# Autodesk Inventor assembly: 09
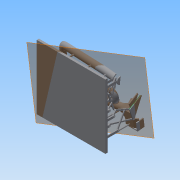
[picture p0: Inventor's stored thumbnail of the model, 180x180]
Saved by Autodesk Inventor 2015 (Build 190159000, 159)
## iProperties
Created: 2018-05-07
Part Number: 09
Document SubType Name: Assembly
Designer: 王博聖
Author: 王博聖
## Documents named in this file (14)
- C:\Users\王博聖\Desktop\0507\09.iam
- C:\Users\王博聖\Desktop\0507\0.ipt
- C:\Users\王博聖\Desktop\0507\1.ipt
- C:\Users\王博聖\Desktop\0507\1-1.ipt
- C:\Users\王博聖\Desktop\0507\1-2.ipt
- C:\Users\王博聖\Desktop\0507\1-3.ipt
- C:\Users\王博聖\Desktop\0507\1-4.ipt
- C:\Users\王博聖\Desktop\0507\2.ipt
- C:\Users\王博聖\Desktop\0507\3.ipt
- C:\Users\王博聖\Desktop\0507\4.ipt
- C:\Users\王博聖\Desktop\0507\5.ipt
- C:\Users\王博聖\Desktop\0507\4456.ipt
- C:\Users\王博聖\Desktop\0507\4444.ipt
- C:\Users\王博聖\Desktop\0507\66666.ipt
## Components (23 placed, 13 different names)
1. 0:1 — 貼合:1, 貼合:2, 貼合:3, 貼合:4, 貼合:5, 貼合:14, 旋轉:1, 齊平:2, 齊平:3, 齊平:5, 齊平:6, 齊平:7, 貼合:29, 齊平:9, 貼合:37, 貼合:38, 貼合:39
2. 1:1 — 貼合:1, 貼合:13, 貼合:25, 貼合:31, 齊平:11
3. 1-1:1 — 貼合:13, 貼合:15, 貼合:24, 貼合:25, 齊平:4, 貼合:33
4. 1-4:1 — 貼合:9, 貼合:20, 貼合:26, 貼合:27, 貼合:35, 貼合:36
5. 2:1 — 貼合:2, 貼合:16, 貼合:23, 貼合:30, 齊平:10
6. 3:1 — 貼合:3, 貼合:14, 貼合:18, 貼合:21, 旋轉:1, 貼合:28, 齊平:8
7. 4:1 — 貼合:4, 貼合:9, 貼合:26
8. 5:1 — 貼合:5, 貼合:19, 貼合:34
9. 1-2:1 — 貼合:15, 貼合:16, 貼合:17, 貼合:22, 貼合:23, 貼合:24, 貼合:32
10. 1-3:1 — 貼合:17, 貼合:18, 貼合:19, 貼合:20, 貼合:21, 貼合:22, 貼合:27
11. 4456:1 — 齊平:2, 齊平:3, 齊平:4, 齊平:5, 齊平:6, 齊平:7
12. 4444:1 — 貼合:32
13. 4444:2 — 貼合:33
14. 4444:3 — 貼合:30, 齊平:10
15. 4444:4 — 貼合:31, 齊平:11
16. 4444:5 — 貼合:29, 齊平:9
17. 4444:6 — 貼合:39
18. 4444:7 — 貼合:34
19. 4444:8 — 貼合:35
20. 4444:9 — 貼合:37
21. 4444:10 — 貼合:38
22. 4444:11 — 貼合:36
23. 66666:1 — 貼合:28, 齊平:8
## Relationships (44: Mate 33, Flush 10, RevoluteJoint 1)
- 貼合:1 [Mate]: 0:1 ↔ 1:1
- 貼合:2 [Mate]: 0:1 ↔ 2:1
- 貼合:3 [Mate]: 0:1 ↔ 3:1
- 貼合:4 [Mate]: 0:1 ↔ 4:1
- 貼合:5 [Mate]: 0:1 ↔ 5:1
- 貼合:9 [Mate]: 1-4:1 ↔ 4:1
- 貼合:13 [Mate]: 1:1 ↔ 1-1:1
- 貼合:14 [Mate]: 0:1 ↔ 3:1
- 貼合:15 [Mate]: 1-1:1 ↔ 1-2:1
- 貼合:16 [Mate]: 2:1 ↔ 1-2:1
- 貼合:17 [Mate]: 1-2:1 ↔ 1-3:1
- 貼合:18 [Mate]: 3:1 ↔ 1-3:1
- 貼合:19 [Mate]: 5:1 ↔ 1-3:1
- 貼合:20 [Mate]: 1-4:1 ↔ 1-3:1
- 貼合:21 [Mate]: 3:1 ↔ 1-3:1
- 貼合:22 [Mate]: 1-2:1 ↔ 1-3:1
- 貼合:23 [Mate]: 2:1 ↔ 1-2:1
- 貼合:24 [Mate]: 1-1:1 ↔ 1-2:1
- 貼合:25 [Mate]: 1:1 ↔ 1-1:1
- 貼合:26 [Mate]: 1-4:1 ↔ 4:1
- 貼合:27 [Mate]: 1-4:1 ↔ 1-3:1
- 旋轉:1 [RevoluteJoint]: 0:1 ↔ 3:1
- 齊平:2 [Flush]: 0:1 ↔ 4456:1
- 齊平:3 [Flush]: 0:1 ↔ 4456:1
- 齊平:4 [Flush]: 1-1:1 ↔ 4456:1
- 齊平:5 [Flush]: 0:1 ↔ 4456:1
- 齊平:6 [Flush] (-23 mm): 0:1 ↔ 4456:1
- 齊平:7 [Flush]: 0:1 ↔ 4456:1
- 貼合:28 [Mate]: 3:1 ↔ 66666:1
- 齊平:8 [Flush]: 3:1 ↔ 66666:1
- 貼合:29 [Mate]: 0:1 ↔ 4444:5
- 齊平:9 [Flush]: 0:1 ↔ 4444:5
- 貼合:30 [Mate]: 2:1 ↔ 4444:3
- 齊平:10 [Flush]: 2:1 ↔ 4444:3
- 貼合:31 [Mate]: 1:1 ↔ 4444:4
- 齊平:11 [Flush]: 1:1 ↔ 4444:4
- 貼合:32 [Mate]: 1-2:1 ↔ 4444:1
- 貼合:33 [Mate]: 1-1:1 ↔ 4444:2
- 貼合:34 [Mate]: 5:1 ↔ 4444:7
- 貼合:35 [Mate]: 1-4:1 ↔ 4444:8
- 貼合:36 [Mate]: 1-4:1 ↔ 4444:11
- 貼合:37 [Mate]: 0:1 ↔ 4444:9
- 貼合:38 [Mate]: 0:1 ↔ 4444:10
- 貼合:39 [Mate]: 0:1 ↔ 4444:6
